# Autodesk Inventor assembly: Arcade
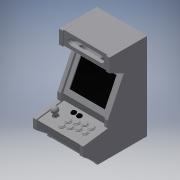
[picture p0: Inventor's stored thumbnail of the model, 180x180]
Saved by Autodesk Inventor 2017 (Build 210142000, 142)
## iProperties
Created: 2019-03-08
Part Number: Arcade
Document SubType Name: Assembly
Designer: Mitch
Author: Mitch
## Documents named in this file (16)
- E:\Youtube Channel\Pojects\Pi Arcade\Mech\Arcade.iam
- E:\Youtube Channel\Pojects\Pi Arcade\Mech\Side Panel.ipt
- E:\Youtube Channel\Pojects\Pi Arcade\Mech\controlBoard.ipt
- E:\Youtube Channel\Pojects\Pi Arcade\Mech\Marque.ipt
- E:\Youtube Channel\Pojects\Pi Arcade\Mech\Top.ipt
- E:\Youtube Channel\Pojects\Pi Arcade\Mech\Back.ipt
- E:\Youtube Channel\Pojects\Pi Arcade\Mech\control front.ipt
- E:\Youtube Channel\Pojects\Pi Arcade\Mech\slant_front.ipt
- E:\Youtube Channel\Pojects\Pi Arcade\Mech\bottom.ipt
- E:\Youtube Channel\Pojects\Pi Arcade\Mech\front_screen_footer.ipt
- E:\Youtube Channel\Pojects\Pi Arcade\Mech\top_slant.ipt
- E:\Youtube Channel\Pojects\Pi Arcade\Mech\screen_holder.ipt
- E:\Youtube Channel\Pojects\Pi Arcade\Mech\screen.ipt
- E:\Youtube Channel\Pojects\Pi Arcade\Mech\small_button.ipt
- E:\Youtube Channel\Pojects\Pi Arcade\Mech\Large_button.ipt
- E:\Youtube Channel\Pojects\Pi Arcade\Mech\Joy_Stick.ipt
## Components (24 placed, 15 different names)
1. Side Panel:1 — Mate:46, Flush:1, Flush:2, Mate:48, Flush:5, Flush:6, Mate:49, Flush:7, Mate:51, Angle:1, Mate:52, Mate:53, Mate:55, Flush:10, Mate:66, Mate:68, Mate:69, Flush:20, Mate:74
2. Side Panel:2 — Mate:47, Flush:4, Flush:8, Flush:18
3. controlBoard:1 — Mate:24, Mate:25, Mate:26, Mate:27, Mate:28, Mate:29, Mate:30, Mate:31, Mate:32, Mate:33, Mate:34, Mate:35, Mate:36, Mate:37, Mate:38, Mate:39, Mate:40, Mate:41, Mate:42, Mate:43, Mate:44, Mate:45, Mate:51, Flush:8, Angle:1, Mate:52, Mate:54, Flush:9, Mate:67, Flush:19
4. Marque:1 — Mate:74, Flush:22
5. Top:1 — Mate:46, Flush:1, Flush:2, Mate:47, Flush:4, Mate:50, Flush:18, Flush:22
6. Back:1 — Mate:49, Mate:50, Flush:7
7. control front:1 — Mate:53, Mate:54, Flush:9, Mate:56
8. slant_front:1 — Mate:55, Mate:56, Flush:10
9. bottom:1 — Mate:48, Flush:5, Flush:6
10. top_slant:1
11. screen_holder:1 — Mate:68, Mate:69, Flush:20, Flush:23, Mate:75, Flush:24
12. screen:1 — Flush:23, Mate:75, Flush:24
13. small_button:1 — Mate:24, Mate:43
14. small_button:2 — Mate:25, Mate:42
15. Large_button:1 — Mate:28, Mate:37
16. Large_button:2 — Mate:29, Mate:34
17. Large_button:3 — Mate:31, Mate:36
18. Large_button:4 — Mate:33, Mate:40
19. Large_button:5 — Mate:26, Mate:41
20. Large_button:6 — Mate:27, Mate:39
21. Large_button:7 — Mate:30, Mate:35
22. Large_button:8 — Mate:32, Mate:38
23. Joy_Stick:1 — Mate:44, Mate:45
24. front_screen_footer:1 — Mate:66, Mate:67, Flush:19
## Relationships (55: Mate 39, Flush 15, Angle 1)
- Mate:24: controlBoard:1 ↔ small_button:1
- Mate:25: controlBoard:1 ↔ small_button:2
- Mate:26: controlBoard:1 ↔ Large_button:5
- Mate:27: controlBoard:1 ↔ Large_button:6
- Mate:28: controlBoard:1 ↔ Large_button:1
- Mate:29: controlBoard:1 ↔ Large_button:2
- Mate:30: controlBoard:1 ↔ Large_button:7
- Mate:31: controlBoard:1 ↔ Large_button:3
- Mate:32: controlBoard:1 ↔ Large_button:8
- Mate:33: controlBoard:1 ↔ Large_button:4
- Mate:34: controlBoard:1 ↔ Large_button:2
- Mate:35: controlBoard:1 ↔ Large_button:7
- Mate:36: controlBoard:1 ↔ Large_button:3
- Mate:37: controlBoard:1 ↔ Large_button:1
- Mate:38: controlBoard:1 ↔ Large_button:8
- Mate:39: controlBoard:1 ↔ Large_button:6
- Mate:40: controlBoard:1 ↔ Large_button:4
- Mate:41: controlBoard:1 ↔ Large_button:5
- Mate:42: controlBoard:1 ↔ small_button:2
- Mate:43: controlBoard:1 ↔ small_button:1
- Mate:44: controlBoard:1 ↔ Joy_Stick:1
- Mate:45: controlBoard:1 ↔ Joy_Stick:1
- Mate:46: Side Panel:1 ↔ Top:1
- Flush:1: Side Panel:1 ↔ Top:1
- Flush:2: Side Panel:1 ↔ Top:1
- Mate:47: Side Panel:2 ↔ Top:1
- Flush:4: Side Panel:2 ↔ Top:1
- Mate:48: Side Panel:1 ↔ bottom:1
- Flush:5: Side Panel:1 ↔ bottom:1
- Flush:6: Side Panel:1 ↔ bottom:1
- Mate:49: Side Panel:1 ↔ Back:1
- Mate:50: Top:1 ↔ Back:1
- Flush:7: Side Panel:1 ↔ Back:1
- Mate:51: Side Panel:1 ↔ controlBoard:1
- Flush:8 (6.35 mm): Side Panel:2 ↔ controlBoard:1
- Angle:1 (8 deg): Side Panel:1 ↔ controlBoard:1
- Mate:52 (-6.35 mm): Side Panel:1 ↔ controlBoard:1
- Mate:53: Side Panel:1 ↔ control front:1
- Mate:54: controlBoard:1 ↔ control front:1
- Flush:9: controlBoard:1 ↔ control front:1
- Mate:55: Side Panel:1 ↔ slant_front:1
- Mate:56: control front:1 ↔ slant_front:1
- Flush:10 (8.7122 mm): Side Panel:1 ↔ slant_front:1
- Flush:18: Side Panel:2 ↔ Top:1
- Mate:66: Side Panel:1 ↔ front_screen_footer:1
- Mate:67: controlBoard:1 ↔ front_screen_footer:1
- Mate:68: Side Panel:1 ↔ screen_holder:1
- Mate:69: Side Panel:1 ↔ screen_holder:1
- Flush:19: controlBoard:1 ↔ front_screen_footer:1
- Flush:20 (12.7 mm): Side Panel:1 ↔ screen_holder:1
- Mate:74: Side Panel:1 ↔ Marque:1
- Flush:22: Marque:1 ↔ Top:1
- Flush:23 (7.1437 mm): screen_holder:1 ↔ screen:1
- Mate:75: screen_holder:1 ↔ screen:1
- Flush:24: screen_holder:1 ↔ screen:1
